# Autodesk Inventor assembly: Lotus_assembly
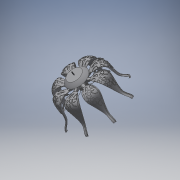
[picture p0: Inventor's stored thumbnail of the model, 180x180]
Saved by Autodesk Inventor 2019 (Build 230136000, 136)
## iProperties
Created: 2019-11-12
Part Number: Lotus_assembly
Document SubType Name: Assembly
Designer: Jorian Brusind
Author: Jorian Brusind
## Documents named in this file (9)
- C:\Users\Jorian Brusind\Documents\GitHub\PersonalProjects\Inventor Projects\Johan\Inventor Files\Lotus_assembly.iam
- C:\Users\Jorian Brusind\Documents\GitHub\PersonalProjects\Inventor Projects\Johan\Inventor Files\Lotus_Petal.ipt
- C:\Users\Jorian Brusind\Documents\GitHub\PersonalProjects\Inventor Projects\Johan\Inventor Files\Ring.ipt
- C:\Users\Jorian Brusind\Documents\GitHub\PersonalProjects\Inventor Projects\Johan\Inventor Files\Leaf.ipt
- C:\Users\Jorian Brusind\Documents\GitHub\PersonalProjects\Inventor Projects\Johan\Inventor Files\inner_ring.ipt
- C:\Users\Jorian Brusind\Documents\GitHub\PersonalProjects\Inventor Projects\Johan\Inventor Files\Innter_petal.ipt
- C:\Users\Jorian Brusind\Documents\GitHub\PersonalProjects\Inventor Projects\Johan\Inventor Files\Threaded_Rod.ipt
- C:\Users\Jorian Brusind\Documents\GitHub\PersonalProjects\Inventor Projects\Johan\Inventor Files\Connector_Rd.ipt
- C:\Users\Jorian Brusind\Documents\GitHub\PersonalProjects\Inventor Projects\Johan\Inventor Files\Hex_Center.ipt
## Components (25 placed, 8 different names)
1. Lotus_Petal:1 — Mate:6, Flush:8, Mate:27
2. Lotus_Petal:2 — Mate:2, Flush:6, Mate:32
3. Lotus_Petal:4 — Mate:4, Flush:1, Mate:25
4. Lotus_Petal:5 — Mate:1, Flush:4, Mate:36
5. Lotus_Petal:6 — Mate:3, Flush:5, Mate:34
6. Lotus_Petal:7 — Mate:5, Flush:7, Mate:29
7. Ring:1 — Mate:1, Mate:2, Mate:3, Mate:4, Mate:5, Mate:6, Mate:7, Mate:8, Flush:1, Flush:2, Flush:3, Flush:4, Flush:5, Flush:6, Flush:7, Flush:8, Mate:9, Mate:10, Mate:11, Mate:12, Mate:19
8. Lotus_Petal:8 — Mate:7, Flush:2, Mate:23
9. Lotus_Petal:9 — Mate:8, Flush:3, Mate:21
10. Leaf:1 — Mate:9, Mate:10, Flush:15
11. inner_ring:1 — Mate:11, Mate:12, Mate:13, Flush:9, Mate:14, Flush:10, Mate:15, Flush:11, Mate:16, Flush:12
12. Innter_petal:1 — Mate:13, Flush:9
13. Innter_petal:2 — Mate:16, Flush:12
14. Innter_petal:5 — Mate:14, Flush:10
15. Innter_petal:6 — Mate:15, Flush:11
16. Threaded_Rod:1 — Mate:19, Flush:15, Mate:37
17. Connector_Rd:1 — Mate:21, Mate:38, Flush:18
18. Connector_Rd:2 — Mate:29, Mate:42, Flush:22
19. Connector_Rd:3 — Mate:34, Mate:40, Flush:20
20. Connector_Rd:5 — Mate:27, Mate:43, Flush:23
21. Connector_Rd:6 — Mate:25, Mate:44, Flush:16
22. Connector_Rd:7 — Mate:23, Mate:45, Flush:17
23. Connector_Rd:8 — Mate:32, Mate:41, Flush:21
24. Connector_Rd:9 — Mate:36, Mate:39, Flush:19
25. Hex_Center:1 — Mate:37, Mate:38, Mate:39, Mate:40, Mate:41, Mate:42, Mate:43, Mate:44, Mate:45, Flush:16, Flush:17, Flush:18, Flush:19, Flush:20, Flush:21, Flush:22, Flush:23
## Relationships (55: Mate 34, Flush 21)
- Mate:1: Lotus_Petal:5 ↔ Ring:1
- Mate:2: Lotus_Petal:2 ↔ Ring:1
- Mate:3: Lotus_Petal:6 ↔ Ring:1
- Mate:4: Lotus_Petal:4 ↔ Ring:1
- Mate:5: Lotus_Petal:7 ↔ Ring:1
- Mate:6: Lotus_Petal:1 ↔ Ring:1
- Mate:7: Ring:1 ↔ Lotus_Petal:8
- Mate:8: Ring:1 ↔ Lotus_Petal:9
- Flush:1: Lotus_Petal:4 ↔ Ring:1
- Flush:2: Ring:1 ↔ Lotus_Petal:8
- Flush:3: Ring:1 ↔ Lotus_Petal:9
- Flush:4: Lotus_Petal:5 ↔ Ring:1
- Flush:5: Lotus_Petal:6 ↔ Ring:1
- Flush:6: Lotus_Petal:2 ↔ Ring:1
- Flush:7: Lotus_Petal:7 ↔ Ring:1
- Flush:8: Lotus_Petal:1 ↔ Ring:1
- Mate:9 (15 mm): Ring:1 ↔ Leaf:1
- Mate:10: Ring:1 ↔ Leaf:1
- Mate:11: Ring:1 ↔ inner_ring:1
- Mate:12 (30 mm): Ring:1 ↔ inner_ring:1
- Mate:13: inner_ring:1 ↔ Innter_petal:1
- Flush:9: inner_ring:1 ↔ Innter_petal:1
- Mate:14: inner_ring:1 ↔ Innter_petal:5
- Flush:10: inner_ring:1 ↔ Innter_petal:5
- Mate:15: inner_ring:1 ↔ Innter_petal:6
- Flush:11: inner_ring:1 ↔ Innter_petal:6
- Mate:16: inner_ring:1 ↔ Innter_petal:2
- Flush:12: inner_ring:1 ↔ Innter_petal:2
- Mate:19: Ring:1 ↔ Threaded_Rod:1
- Flush:15 (-10 mm): Leaf:1 ↔ Threaded_Rod:1
- Mate:21: Lotus_Petal:9 ↔ Connector_Rd:1
- Mate:23: Lotus_Petal:8 ↔ Connector_Rd:7
- Mate:25: Lotus_Petal:4 ↔ Connector_Rd:6
- Mate:27: Lotus_Petal:1 ↔ Connector_Rd:5
- Mate:29: Lotus_Petal:7 ↔ Connector_Rd:2
- Mate:32: Lotus_Petal:2 ↔ Connector_Rd:8
- Mate:34: Lotus_Petal:6 ↔ Connector_Rd:3
- Mate:36: Lotus_Petal:5 ↔ Connector_Rd:9
- Mate:37: Threaded_Rod:1 ↔ Hex_Center:1
- Mate:38: Connector_Rd:1 ↔ Hex_Center:1
- Mate:39: Connector_Rd:9 ↔ Hex_Center:1
- Mate:40: Connector_Rd:3 ↔ Hex_Center:1
- Mate:41: Connector_Rd:8 ↔ Hex_Center:1
- Mate:42: Connector_Rd:2 ↔ Hex_Center:1
- Mate:43: Connector_Rd:5 ↔ Hex_Center:1
- Mate:44: Connector_Rd:6 ↔ Hex_Center:1
- Mate:45: Connector_Rd:7 ↔ Hex_Center:1
- Flush:16 (1.15 mm): Connector_Rd:6 ↔ Hex_Center:1
- Flush:17 (-1.15 mm): Connector_Rd:7 ↔ Hex_Center:1
- Flush:18 (1.15 mm): Connector_Rd:1 ↔ Hex_Center:1
- Flush:19 (1.15 mm): Connector_Rd:9 ↔ Hex_Center:1
- Flush:20 (1.15 mm): Connector_Rd:3 ↔ Hex_Center:1
- Flush:21 (1.15 mm): Connector_Rd:8 ↔ Hex_Center:1
- Flush:22 (-1.15 mm): Connector_Rd:2 ↔ Hex_Center:1
- Flush:23 (1.15 mm): Connector_Rd:5 ↔ Hex_Center:1
